# Autodesk Inventor assembly: Custom Slewing
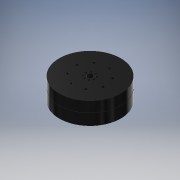
[picture p0: Inventor's stored thumbnail of the model, 180x180]
Saved by Autodesk Inventor 2017 (Build 210142000, 142)
## iProperties
Created: 2019-11-06
Part Number: Custom Slewing
Document SubType Name: Assembly
Designer: Dell
Author: Dell
## Documents named in this file (6)
- C:\Users\Dell\Documents\GitHub\tr2\Actuator 2.0\Custom Slewing.iam
- C:\Users\Dell\Documents\GitHub\tr2\Actuator 2.0\51205.ipt
- C:\Users\Dell\Documents\GitHub\tr2\Actuator 2.0\AXK80105 2AS.ipt
- C:\Users\Dell\Documents\GitHub\tr2\Actuator 2.0\CS01.ipt
- C:\Users\Dell\Documents\GitHub\tr2\Actuator 2.0\CS02.ipt
- C:\Users\Dell\Documents\GitHub\tr2\Actuator 2.0\CS03.ipt
## Components (5 placed, 5 different names)
1. 51205:1 — Mate:1, Mate:2, Mate:3, Mate:4, Mate:5
2. AXK80105 2AS:1 — Mate:1, Mate:6, Mate:8
3. CS01:1 — Mate:2, Mate:3, Mate:7, Mate:9
4. CS02:1 — Mate:4, Mate:5, Mate:6
5. CS03:1 — Mate:7, Mate:8, Mate:9
## Relationships (9: Mate 9)
- Mate:1: 51205:1 ↔ AXK80105 2AS:1
- Mate:2: 51205:1 ↔ CS01:1
- Mate:3: 51205:1 ↔ CS01:1
- Mate:4: 51205:1 ↔ CS02:1
- Mate:5: 51205:1 ↔ CS02:1
- Mate:6: AXK80105 2AS:1 ↔ CS02:1
- Mate:7: CS01:1 ↔ CS03:1
- Mate:8: AXK80105 2AS:1 ↔ CS03:1
- Mate:9: CS01:1 ↔ CS03:1
